# Autodesk Inventor assembly: цепь
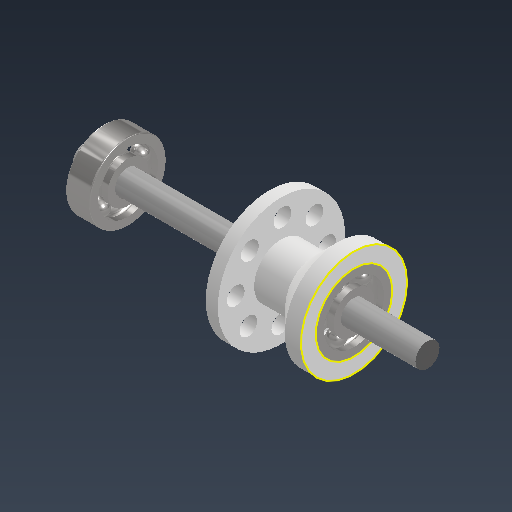
[picture p0: Inventor's stored thumbnail of the model, 512x512]
Saved by Autodesk Inventor 2026 (Build 300175000, 175)
## iProperties
Created: 2024-07-09
Part Number: цепь
Document SubType Name: Assembly
Designer: Phantom
Author: Phantom
## Documents named in this file (4)
- C:\Users\GameHD\Desktop\Phantom 16950\цепь.iam
- C:\Users\GameHD\Desktop\Phantom 16950\втулка для подш 2 часть.ipt
- C:\Users\GameHD\Desktop\Phantom 16950\Деталь_64.ipt
- C:\Users\GameHD\Desktop\Phantom 16950\BS 290 SKF - SKF 626-RZ.ipt
## Components (4 placed, 3 different names)
1. втулка для подш 2 часть:1 — Совмещение:20, Совмещение:23
2. Деталь_64:1 — Совмещение:19, Совмещение:21, Совмещение:23
3. BS 290 SKF - SKF 626-RZ:1 — Совмещение:20, Совмещение:21
4. BS 290 SKF - SKF 626-RZ:2 — Совмещение:19
## Relationships (4: Mate 4)
- Совмещение:19 [Mate]: Деталь_64:1 ↔ BS 290 SKF - SKF 626-RZ:2
- Совмещение:20 [Mate]: втулка для подш 2 часть:1 ↔ BS 290 SKF - SKF 626-RZ:1
- Совмещение:21 [Mate]: Деталь_64:1 ↔ BS 290 SKF - SKF 626-RZ:1
- Совмещение:23 [Mate]: втулка для подш 2 часть:1 ↔ Деталь_64:1
